# Autodesk Inventor assembly: 000-roller-hand-v2
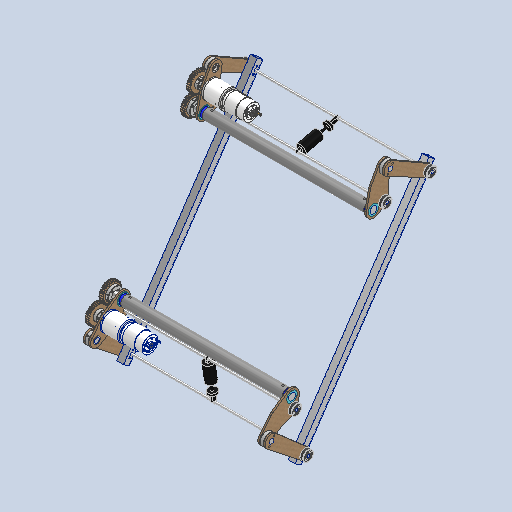
[picture p0: Inventor's stored thumbnail of the model, 512x512]
Saved by Autodesk Inventor 2025.1 (Build 291241000, 241)
## iProperties
Created: 2024-10-06
Part Number: 000-roller-hand-v2
Document SubType Name: Assembly
Designer: haruy
Author: haruy
## Documents named in this file (3)
- C:\Users\haruy\Documents\ロボコン\NHK2025\cad\nagahisa\hand\roller\000-roller-hand-v2.iam
- C:\Users\haruy\Documents\ロボコン\NHK2025\cad\nagahisa\hand\roller\roller-hand-v2-P.iam
- C:\Users\haruy\Documents\ロボコン\NHK2025\cad\nagahisa\hand\roller\roller-hand-v1-roller.ipt
## Components (3 placed, 2 different names)
1. roller-hand-v2-P:1 [sub-assembly] — 挿入:1, 挿入:2
2. roller-hand-v1-roller:1 — 挿入:1
3. roller-hand-v1-roller:2 — 挿入:2
## Relationships (2: Insert 2)
- 挿入:1 [Insert]: roller-hand-v2-P:1 ↔ roller-hand-v1-roller:1
- 挿入:2 [Insert]: roller-hand-v2-P:1 ↔ roller-hand-v1-roller:2
